# Autodesk Inventor assembly: Hopper Driver Holder
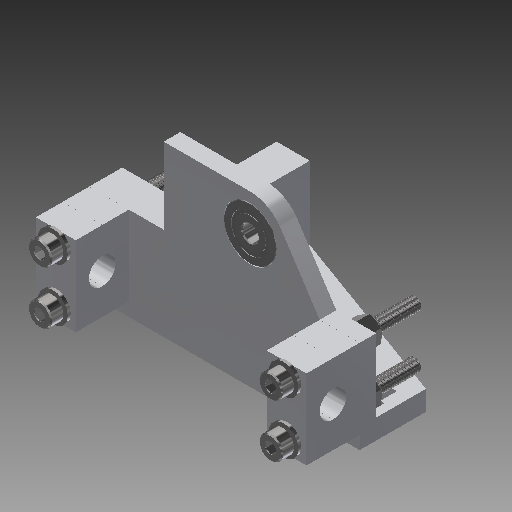
[picture p0: Inventor's stored thumbnail of the model, 512x512]
Saved by Autodesk Inventor 2018 (Build 220112000, 112)
## iProperties
Created: 2017-09-19
Part Number: Hopper Driver Holder
Document SubType Name: Assembly
Designer: Gabriel Smolnycki
Author: Gabriel Smolnycki
## Documents named in this file (7)
- E:\planb\mechanics\Subassemblies\Hopper Driver Holder assy.iam
- E:\planb\mechanics\Hopper\Hopper Rod Clamp.ipt
- E:\planb\mechanics\Hardware\5x16 SS Ball Bearing (6153K150).ipt
- E:\planb\mechanics\Hopper\Hopper Smooth Rod Clamp.ipt
- E:\planb\mechanics\Hardware\M4x40 SS SHCS.ipt
- E:\planb\mechanics\Hardware\M4 SS Washer.ipt
- E:\planb\mechanics\Hardware\M4 SS Locknut.ipt
## Components (16 placed, 6 different names)
1. Hopper Rod Clamp:1 — Insert:1, Insert:2, Insert:3, Insert:10, Insert:11, Insert:12, Insert:13
2. 5x16 SS Ball Bearing (6153K150):1 — Insert:1
3. Hopper Smooth Rod Clamp:1 — Insert:2, Insert:3, Insert:4, Insert:5
4. Hopper Smooth Rod Clamp:2 — Insert:4, Insert:5, Insert:6, Insert:7
5. M4x40 SS SHCS:1 — Insert:9
6. M4x40 SS SHCS:2 — Insert:8
7. M4 SS Washer:1 — Insert:7, Insert:9
8. M4 SS Washer:2 — Insert:6, Insert:8
9. M4 SS Locknut:1 — Insert:11
10. M4 SS Locknut:2 — Insert:10
11. Hopper Smooth Rod Clamp:3 — Insert:14, Insert:15, Insert:16, Insert:17
12. Hopper Smooth Rod Clamp:4 — Insert:12, Insert:13, Insert:14, Insert:15
13. M4x40 SS SHCS:3 — Insert:19
14. M4x40 SS SHCS:4 — Insert:18
15. M4 SS Washer:3 — Insert:16, Insert:18
16. M4 SS Washer:4 — Insert:17, Insert:19
## Relationships (19: Insert 19)
- Insert:1: Hopper Rod Clamp:1 ↔ 5x16 SS Ball Bearing (6153K150):1
- Insert:2: Hopper Rod Clamp:1 ↔ Hopper Smooth Rod Clamp:1
- Insert:3: Hopper Rod Clamp:1 ↔ Hopper Smooth Rod Clamp:1
- Insert:4: Hopper Smooth Rod Clamp:1 ↔ Hopper Smooth Rod Clamp:2
- Insert:5: Hopper Smooth Rod Clamp:1 ↔ Hopper Smooth Rod Clamp:2
- Insert:6: Hopper Smooth Rod Clamp:2 ↔ M4 SS Washer:2
- Insert:7: Hopper Smooth Rod Clamp:2 ↔ M4 SS Washer:1
- Insert:8: M4x40 SS SHCS:2 ↔ M4 SS Washer:2
- Insert:9: M4x40 SS SHCS:1 ↔ M4 SS Washer:1
- Insert:10: Hopper Rod Clamp:1 ↔ M4 SS Locknut:2
- Insert:11: Hopper Rod Clamp:1 ↔ M4 SS Locknut:1
- Insert:12: Hopper Rod Clamp:1 ↔ Hopper Smooth Rod Clamp:4
- Insert:13: Hopper Rod Clamp:1 ↔ Hopper Smooth Rod Clamp:4
- Insert:14: Hopper Smooth Rod Clamp:3 ↔ Hopper Smooth Rod Clamp:4
- Insert:15: Hopper Smooth Rod Clamp:3 ↔ Hopper Smooth Rod Clamp:4
- Insert:16: Hopper Smooth Rod Clamp:3 ↔ M4 SS Washer:3
- Insert:17: Hopper Smooth Rod Clamp:3 ↔ M4 SS Washer:4
- Insert:18: M4x40 SS SHCS:4 ↔ M4 SS Washer:3
- Insert:19: M4x40 SS SHCS:3 ↔ M4 SS Washer:4
